# Autodesk Inventor assembly: アーム2
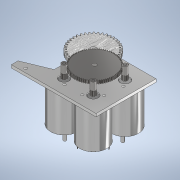
[picture p0: Inventor's stored thumbnail of the model, 180x180]
Saved by Autodesk Inventor 2020.2 (Build 242310000, 310)
## iProperties
Created: 2020-03-16
Part Number: アーム2
Document SubType Name: Assembly
Designer: aoyam
Author: aoyam
## Documents named in this file (5)
- C:\Users\aoyam\Desktop\SRDC_local\Inventor\二年機\インナー4層丙\アーム\アーム2.iam
- C:\Users\aoyam\Desktop\SRDC_local\Inventor\二年機\インナー4層丙\アーム\モーターマウント.ipt
- C:\Users\aoyam\Desktop\SRDC_local\Inventor\二年機\インナー4層丙\汎用部品\マブチRS380アーム用.iam
- C:\Users\aoyam\Desktop\SRDC_local\Inventor\二年機\インナー4層丙\アーム\アーム用初段.iam
- C:\Users\aoyam\Desktop\SRDC_local\Inventor\二年機\インナー4層丙\アーム\アーム用2段.iam
## Components (6 placed, 4 different names)
1. モーターマウント:1 — 挿入:1, メイト:1, 挿入:2, メイト:2, 挿入:3, メイト:3, メイト:4, メイト:5
2. マブチRS380アーム用:1 [sub-assembly] — 挿入:1, メイト:1
3. マブチRS380アーム用:2 [sub-assembly] — 挿入:2, メイト:2
4. マブチRS380アーム用:3 [sub-assembly] — 挿入:3, メイト:3
5. アーム用初段:1 [sub-assembly] — メイト:4
6. アーム用2段:1 [sub-assembly] — メイト:5
## Relationships (8: Mate 5, Insert 3)
- 挿入:1 [Insert]: モーターマウント:1 ↔ マブチRS380アーム用:1
- メイト:1 [Mate]: モーターマウント:1 ↔ マブチRS380アーム用:1
- 挿入:2 [Insert]: モーターマウント:1 ↔ マブチRS380アーム用:2
- メイト:2 [Mate]: モーターマウント:1 ↔ マブチRS380アーム用:2
- 挿入:3 [Insert]: モーターマウント:1 ↔ マブチRS380アーム用:3
- メイト:3 [Mate]: モーターマウント:1 ↔ マブチRS380アーム用:3
- メイト:4 [Mate]: モーターマウント:1 ↔ アーム用初段:1
- メイト:5 [Mate]: モーターマウント:1 ↔ アーム用2段:1
